# Autodesk Inventor assembly: Gearbox Handle
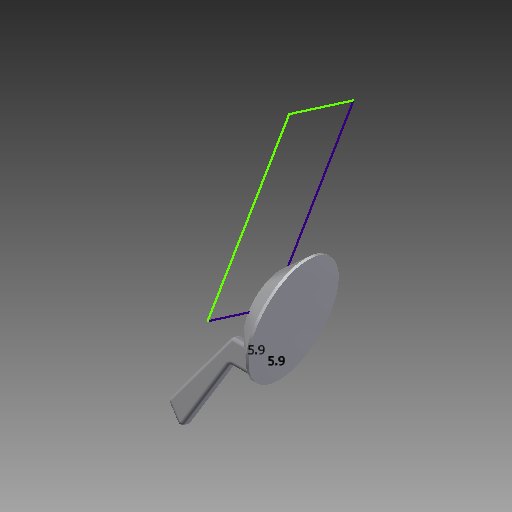
[picture p0: Inventor's stored thumbnail of the model, 512x512]
Saved by Autodesk Inventor 2018 (Build 220112000, 112)
## iProperties
Created: 2017-08-15
Part Number: Gearbox Handle
Document SubType Name: Assembly
Designer: M227562
Author: M227562
## Documents named in this file (3)
- C:\Users\P301319\Documents\GitHub\CNC-Lathe-CAD\Gearbox Handle and other bits\Gearbox Handle.iam
- C:\Users\P301319\Documents\GitHub\CNC-Lathe-CAD\Gearbox Handle and other bits\Handle Gearbox.ipt
- C:\Users\P301319\Documents\GitHub\CNC-Lathe-CAD\Gearbox Handle and other bits\Handle Gearbox handle.ipt
## Components (2 placed, 2 different names)
1. Handle Gearbox:1 — Rigid:1
2. Handle Gearbox handle:1 — Rigid:1
## Relationships (1: WeldJoint 1)
- Rigid:1 [WeldJoint] (-12 mm): Handle Gearbox:1 ↔ Handle Gearbox handle:1
